# Autodesk Inventor assembly: actor-re-actor
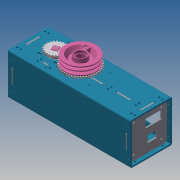
[picture p0: Inventor's stored thumbnail of the model, 180x180]
Saved by Autodesk Inventor 2017 (Build 210142000, 142)
## iProperties
Part Number: actor-re-actor
Material: Genérico
Document SubType Name: Assembly
Designer: FABLAB
Author: FABLAB
## Documents named in this file (5)
- C:\Users\FABLAB\Dropbox\E\Caja Motriz\actor-re-actor.iam
- C:\Users\FABLAB\Dropbox\E\Caja Motriz\CaseC.iam
- C:\Users\FABLAB\Dropbox\E\Caja Motriz\transmision Engranajes\Potencia.iam
- C:\Users\FABLAB\Dropbox\E\Caja Motriz\transmision Engranajes\Plato Carrete-doble B.iam
- C:\Users\FABLAB\Dropbox\E\Caja Motriz\actor-re-actor\Design Accelerator\Engranajes rectos1.iam
## Components (4 placed, 4 different names)
1. CaseC:1 [sub-assembly] — Coincidencia:1, Coincidencia:4
2. Potencia:1 [sub-assembly] — Coincidencia:1, Coincidencia:2, Coincidencia:3
3. Plato Carrete-doble B:1 [sub-assembly] — Coincidencia:4, Coincidencia:5, Coincidencia:6
4. Engranajes rectos:1 [sub-assembly]
## Relationships (6: Mate 6)
- Coincidencia:1 [Mate] (2 mm): CaseC:1 ↔ Potencia:1
- Coincidencia:2 [Mate]: Potencia:1
- Coincidencia:3 [Mate]: Potencia:1
- Coincidencia:4 [Mate] (5 mm): CaseC:1 ↔ Plato Carrete-doble B:1
- Coincidencia:5 [Mate]: Plato Carrete-doble B:1
- Coincidencia:6 [Mate] (72 mm): Plato Carrete-doble B:1
